# Autodesk Inventor assembly: MK4n Master Structure
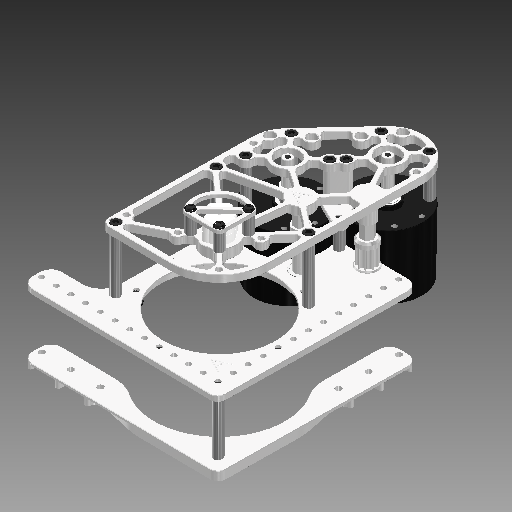
[picture p0: Inventor's stored thumbnail of the model, 512x512]
Saved by Autodesk Inventor 2025 (Build 290162010, 162A)
## iProperties
Created: 2024-07-31
Part Number: MK4n Master Structure
Document SubType Name: Assembly
Designer: rohan
Author: rohan
## Documents named in this file (27)
- D:\ultimate-hecker\Computer-Aided-Design\FRC-Offseason-Design-Training\Parts Library\Drivetrains\Swerve Modules\MK4n\MK4n Master Structure.iam
- D:\ultimate-hecker\Computer-Aided-Design\FRC-Offseason-Design-Training\Parts Library\Drivetrains\Swerve Modules\MK4i\MK4i Wheel Guard.ipt
- D:\ultimate-hecker\Computer-Aided-Design\FRC-Offseason-Design-Training\Parts Library\Drivetrains\Swerve Modules\MK4n\MK4n Midsection.ipt
- D:\ultimate-hecker\Computer-Aided-Design\FRC-Offseason-Design-Training\Parts Library\Drivetrains\Swerve Modules\MK4n\MK4n Motor Mount.ipt
- D:\ultimate-hecker\Computer-Aided-Design\FRC-Offseason-Design-Training\Parts Library\Hardware\Spacers\Spacers & Standoffs\Aluminum Unthreaded Spacer (No. 10 x 1.875Lg x 0.313OD).ipt
- D:\ultimate-hecker\Computer-Aided-Design\FRC-Offseason-Design-Training\Parts Library\Hardware\Spacers\Spacers & Standoffs.ipt
- D:\ultimate-hecker\Computer-Aided-Design\FRC-Offseason-Design-Training\Parts Library\Hardware\Fasteners\Machine Screws\10-32 UNFx2.25 Socket Head Cap Screw.ipt
- D:\ultimate-hecker\Computer-Aided-Design\FRC-Offseason-Design-Training\Parts Library\Hardware\Fasteners\Machine Screws.ipt
- D:\ultimate-hecker\Computer-Aided-Design\FRC-Offseason-Design-Training\Parts Library\Hardware\Spacers\Spacers & Standoffs\Aluminum Unthreaded Spacer (No. 10 x 1.125Lg x 0.313OD).ipt
- D:\ultimate-hecker\Computer-Aided-Design\FRC-Offseason-Design-Training\Parts Library\Hardware\Spacers\Spacers & Standoffs\Aluminum Unthreaded Spacer (No. 10 x 0.625Lg x 0.313OD).ipt
- D:\ultimate-hecker\Computer-Aided-Design\FRC-Offseason-Design-Training\Parts Library\Drivetrains\Swerve Modules\MK4n\MK4n Double Spacer Adapter.ipt
- D:\ultimate-hecker\Computer-Aided-Design\FRC-Offseason-Design-Training\Parts Library\Drivetrains\Swerve Modules\MK4n\MK4n Double Spacer.ipt
- D:\ultimate-hecker\Computer-Aided-Design\FRC-Offseason-Design-Training\Parts Library\Motors\FRC\NEO.ipt
- D:\ultimate-hecker\Computer-Aided-Design\FRC-Offseason-Design-Training\Parts Library\Hardware\Fasteners\Machine Screws\10-32 UNFx1.5 Socket Head Cap Screw.ipt
- D:\ultimate-hecker\Computer-Aided-Design\FRC-Offseason-Design-Training\Parts Library\Hardware\Fasteners\Machine Screws\10-32 UNFx1 Socket Head Cap Screw.ipt
- D:\ultimate-hecker\Computer-Aided-Design\FRC-Offseason-Design-Training\Parts Library\Power Transfer\Bearings and Bushings\Bearings\R188ZZ Bearing.ipt
- D:\ultimate-hecker\Computer-Aided-Design\FRC-Offseason-Design-Training\Parts Library\Drivetrains\Swerve Modules\MK4i\MK4i Steering Shaft Spacer.ipt
- D:\ultimate-hecker\Computer-Aided-Design\FRC-Offseason-Design-Training\Parts Library\Drivetrains\Swerve Modules\MK4i\MK4i Steering Shaft.ipt
- D:\ultimate-hecker\Computer-Aided-Design\FRC-Offseason-Design-Training\Parts Library\Power Transfer\Bearings and Bushings\Bearings\688 Bearing.ipt
- D:\ultimate-hecker\Computer-Aided-Design\FRC-Offseason-Design-Training\Parts Library\Hardware\Spacers\Spacers & Standoffs\SDS Neo Shaft Spacer 0.5mm.ipt
- D:\ultimate-hecker\Computer-Aided-Design\FRC-Offseason-Design-Training\Parts Library\Hardware\Spacers\Spacers & Standoffs\SDS Neo Shaft Spacer 0.437.ipt
- D:\ultimate-hecker\Computer-Aided-Design\FRC-Offseason-Design-Training\Parts Library\Drivetrains\Swerve Modules\MK4i\MK4i Drive Shaft Idler.ipt
- D:\ultimate-hecker\Computer-Aided-Design\FRC-Offseason-Design-Training\Parts Library\Hardware\Spacers\Spacers & Standoffs\Aluminum Unthreaded Spacer (No. 10 x 0.563Lg x 0.313OD).ipt
- D:\ultimate-hecker\Computer-Aided-Design\FRC-Offseason-Design-Training\Parts Library\Drivetrains\Swerve Modules\MK4i\MK4i Encoder Cover.ipt
- D:\ultimate-hecker\Computer-Aided-Design\FRC-Offseason-Design-Training\Parts Library\Electronics\FRC\Sensors\CTRE Mag Encoder.ipt
- D:\ultimate-hecker\Computer-Aided-Design\FRC-Offseason-Design-Training\Parts Library\Hardware\Fasteners\Machine Screws\8-32 UNCx0.875 Button Head Cap Screw.ipt
- D:\ultimate-hecker\Computer-Aided-Design\FRC-Offseason-Design-Training\Parts Library\Hardware\Fasteners\Machine Screws\10-32 UNFx0.25 Button Head Cap Screw.ipt
## Components (49 placed, 24 different names)
1. MK4i Wheel Guard:1 — Insert:1, Insert:11, Flush:1
2. MK4n Midsection:1 — Insert:2, Insert:3, Insert:5, Insert:7, Insert:19, Insert:32, Insert:33, Insert:37, Flush:1, Insert:50, Insert:51, Insert:52, Insert:53, Insert:54
3. MK4n Motor Mount:1 — Insert:4, Insert:6, Insert:8, Insert:9, Insert:10, Insert:12, Insert:13, Insert:14, Insert:15, Insert:20, Insert:21, Insert:26, Insert:27, Insert:28, Insert:29, Insert:30, Insert:31, Insert:34, Insert:38, Insert:40, Insert:41, Insert:42, Insert:45, Insert:46
4. Aluminum Unthreaded Spacer (No. 10 x 1.875Lg x 0.313OD):1 — Insert:3, Insert:4
5. Aluminum Unthreaded Spacer (No. 10 x 1.875Lg x 0.313OD):2 — Insert:5, Insert:6
6. Aluminum Unthreaded Spacer (No. 10 x 1.875Lg x 0.313OD):3 — Insert:1, Insert:2
7. Aluminum Unthreaded Spacer (No. 10 x 1.875Lg x 0.313OD):6 — Insert:7
8. 10-32 UNFx2.25 Socket Head Cap Screw:1 — Insert:8
9. 10-32 UNFx2.25 Socket Head Cap Screw:2 — Insert:9
10. 10-32 UNFx2.25 Socket Head Cap Screw:3 — Insert:11
11. 10-32 UNFx2.25 Socket Head Cap Screw:4 — Insert:10
12. Aluminum Unthreaded Spacer (No. 10 x 1.125Lg x 0.313OD):7 — Insert:12
13. Aluminum Unthreaded Spacer (No. 10 x 1.125Lg x 0.313OD):8 — Insert:14, Insert:25
14. Aluminum Unthreaded Spacer (No. 10 x 1.125Lg x 0.313OD):9 — Insert:13, Insert:22
15. Aluminum Unthreaded Spacer (No. 10 x 1.125Lg x 0.313OD):10 — Insert:15, Insert:24
16. Aluminum Unthreaded Spacer (No. 10 x 0.625Lg x 0.313OD):11 — Insert:18, Insert:19
17. MK4n Double Spacer Adapter:1 — Insert:16, Insert:17, Insert:18, Insert:23
18. MK4n Double Spacer:1 — Insert:16, Insert:17, Insert:20, Insert:21
19. NEO:1 — Insert:22, Insert:23, Insert:35
20. NEO:2 — Insert:24, Insert:25, Insert:36
21. 10-32 UNFx1.5 Socket Head Cap Screw:5 — Insert:30
22. 10-32 UNFx1.5 Socket Head Cap Screw:6 — Insert:31
23. 10-32 UNFx1.5 Socket Head Cap Screw:7 — Insert:28
24. 10-32 UNFx1.5 Socket Head Cap Screw:8 — Insert:29
25. 10-32 UNFx1.5 Socket Head Cap Screw:9 — Insert:26
26. 10-32 UNFx1.5 Socket Head Cap Screw:10 — Insert:27
27. 10-32 UNFx1 Socket Head Cap Screw:11 — Insert:32
28. R188ZZ Bearing:1 — Insert:33, Mate:1
29. MK4i Steering Shaft Spacer:1 — Mate:2
30. MK4i Steering Shaft:1 — Mate:1, Mate:2
31. 688 Bearing:1 — Insert:34
32. SDS Neo Shaft Spacer 0.5mm:12 — Insert:35
33. SDS Neo Shaft Spacer 0.437:13 — Insert:36
34. 688 Bearing:2 — Insert:37, Insert:39
35. 688 Bearing:3 — Insert:38
36. MK4i Drive Shaft Idler:1 — Insert:39
37. Aluminum Unthreaded Spacer (No. 10 x 0.563Lg x 0.313OD):17 — Insert:42
38. Aluminum Unthreaded Spacer (No. 10 x 0.563Lg x 0.313OD):18 — Insert:41, Insert:43
39. Aluminum Unthreaded Spacer (No. 10 x 0.563Lg x 0.313OD):19 — Insert:40, Insert:44
40. MK4i Encoder Cover:1 — Insert:43, Insert:44, Insert:47, Insert:48, Insert:49
41. CTRE Mag Encoder:1 — Insert:45, Insert:46
42. 8-32 UNCx0.875 Button Head Cap Screw:12 — Insert:49
43. 8-32 UNCx0.875 Button Head Cap Screw:13 — Insert:48
44. 8-32 UNCx0.875 Button Head Cap Screw:14 — Insert:47
45. 10-32 UNFx0.25 Button Head Cap Screw:15 — Insert:50
46. 10-32 UNFx0.25 Button Head Cap Screw:16 — Insert:52
47. 10-32 UNFx0.25 Button Head Cap Screw:17 — Insert:54
48. 10-32 UNFx0.25 Button Head Cap Screw:18 — Insert:51
49. 10-32 UNFx0.25 Button Head Cap Screw:19 — Insert:53
## Relationships (57: Insert 54, Mate 2, Flush 1)
- Insert:1: MK4i Wheel Guard:1 ↔ Aluminum Unthreaded Spacer (No. 10 x 1.875Lg x 0.313OD):3
- Insert:2: MK4n Midsection:1 ↔ Aluminum Unthreaded Spacer (No. 10 x 1.875Lg x 0.313OD):3
- Insert:3: MK4n Midsection:1 ↔ Aluminum Unthreaded Spacer (No. 10 x 1.875Lg x 0.313OD):1
- Insert:4: MK4n Motor Mount:1 ↔ Aluminum Unthreaded Spacer (No. 10 x 1.875Lg x 0.313OD):1
- Insert:5: MK4n Midsection:1 ↔ Aluminum Unthreaded Spacer (No. 10 x 1.875Lg x 0.313OD):2
- Insert:6: MK4n Motor Mount:1 ↔ Aluminum Unthreaded Spacer (No. 10 x 1.875Lg x 0.313OD):2
- Insert:7: MK4n Midsection:1 ↔ Aluminum Unthreaded Spacer (No. 10 x 1.875Lg x 0.313OD):6
- Insert:8: MK4n Motor Mount:1 ↔ 10-32 UNFx2.25 Socket Head Cap Screw:1
- Insert:9: MK4n Motor Mount:1 ↔ 10-32 UNFx2.25 Socket Head Cap Screw:2
- Insert:10: MK4n Motor Mount:1 ↔ 10-32 UNFx2.25 Socket Head Cap Screw:4
- Insert:11: MK4i Wheel Guard:1 ↔ 10-32 UNFx2.25 Socket Head Cap Screw:3
- Insert:12: MK4n Motor Mount:1 ↔ Aluminum Unthreaded Spacer (No. 10 x 1.125Lg x 0.313OD):7
- Insert:13: MK4n Motor Mount:1 ↔ Aluminum Unthreaded Spacer (No. 10 x 1.125Lg x 0.313OD):9
- Insert:14: MK4n Motor Mount:1 ↔ Aluminum Unthreaded Spacer (No. 10 x 1.125Lg x 0.313OD):8
- Insert:15: MK4n Motor Mount:1 ↔ Aluminum Unthreaded Spacer (No. 10 x 1.125Lg x 0.313OD):10
- Insert:16: MK4n Double Spacer Adapter:1 ↔ MK4n Double Spacer:1
- Insert:17: MK4n Double Spacer Adapter:1 ↔ MK4n Double Spacer:1
- Insert:18: Aluminum Unthreaded Spacer (No. 10 x 0.625Lg x 0.313OD):11 ↔ MK4n Double Spacer Adapter:1
- Insert:19: MK4n Midsection:1 ↔ Aluminum Unthreaded Spacer (No. 10 x 0.625Lg x 0.313OD):11
- Insert:20: MK4n Motor Mount:1 ↔ MK4n Double Spacer:1
- Insert:21: MK4n Motor Mount:1 ↔ MK4n Double Spacer:1
- Insert:22: Aluminum Unthreaded Spacer (No. 10 x 1.125Lg x 0.313OD):9 ↔ NEO:1
- Insert:23: MK4n Double Spacer Adapter:1 ↔ NEO:1
- Insert:24: Aluminum Unthreaded Spacer (No. 10 x 1.125Lg x 0.313OD):10 ↔ NEO:2
- Insert:25: Aluminum Unthreaded Spacer (No. 10 x 1.125Lg x 0.313OD):8 ↔ NEO:2
- Insert:26: MK4n Motor Mount:1 ↔ 10-32 UNFx1.5 Socket Head Cap Screw:9
- Insert:27: MK4n Motor Mount:1 ↔ 10-32 UNFx1.5 Socket Head Cap Screw:10
- Insert:28: MK4n Motor Mount:1 ↔ 10-32 UNFx1.5 Socket Head Cap Screw:7
- Insert:29: MK4n Motor Mount:1 ↔ 10-32 UNFx1.5 Socket Head Cap Screw:8
- Insert:30: MK4n Motor Mount:1 ↔ 10-32 UNFx1.5 Socket Head Cap Screw:5
- Insert:31: MK4n Motor Mount:1 ↔ 10-32 UNFx1.5 Socket Head Cap Screw:6
- Insert:32: MK4n Midsection:1 ↔ 10-32 UNFx1 Socket Head Cap Screw:11
- Insert:33: MK4n Midsection:1 ↔ R188ZZ Bearing:1
- Insert:34: MK4n Motor Mount:1 ↔ 688 Bearing:1
- Mate:1: R188ZZ Bearing:1 ↔ MK4i Steering Shaft:1
- Mate:2: MK4i Steering Shaft Spacer:1 ↔ MK4i Steering Shaft:1
- Insert:35: NEO:1 ↔ SDS Neo Shaft Spacer 0.5mm:12
- Insert:36: NEO:2 ↔ SDS Neo Shaft Spacer 0.437:13
- Insert:37: MK4n Midsection:1 ↔ 688 Bearing:2
- Insert:38: MK4n Motor Mount:1 ↔ 688 Bearing:3
- Insert:39: 688 Bearing:2 ↔ MK4i Drive Shaft Idler:1
- Insert:40: MK4n Motor Mount:1 ↔ Aluminum Unthreaded Spacer (No. 10 x 0.563Lg x 0.313OD):19
- Insert:41: MK4n Motor Mount:1 ↔ Aluminum Unthreaded Spacer (No. 10 x 0.563Lg x 0.313OD):18
- Insert:42: MK4n Motor Mount:1 ↔ Aluminum Unthreaded Spacer (No. 10 x 0.563Lg x 0.313OD):17
- Insert:43: Aluminum Unthreaded Spacer (No. 10 x 0.563Lg x 0.313OD):18 ↔ MK4i Encoder Cover:1
- Flush:1: MK4i Wheel Guard:1 ↔ MK4n Midsection:1
- Insert:44: Aluminum Unthreaded Spacer (No. 10 x 0.563Lg x 0.313OD):19 ↔ MK4i Encoder Cover:1
- Insert:45: MK4n Motor Mount:1 ↔ CTRE Mag Encoder:1
- Insert:46: MK4n Motor Mount:1 ↔ CTRE Mag Encoder:1
- Insert:47: MK4i Encoder Cover:1 ↔ 8-32 UNCx0.875 Button Head Cap Screw:14
- Insert:48: MK4i Encoder Cover:1 ↔ 8-32 UNCx0.875 Button Head Cap Screw:13
- Insert:49: MK4i Encoder Cover:1 ↔ 8-32 UNCx0.875 Button Head Cap Screw:12
- Insert:50: MK4n Midsection:1 ↔ 10-32 UNFx0.25 Button Head Cap Screw:15
- Insert:51: MK4n Midsection:1 ↔ 10-32 UNFx0.25 Button Head Cap Screw:18
- Insert:52: MK4n Midsection:1 ↔ 10-32 UNFx0.25 Button Head Cap Screw:16
- Insert:53: MK4n Midsection:1 ↔ 10-32 UNFx0.25 Button Head Cap Screw:19
- Insert:54: MK4n Midsection:1 ↔ 10-32 UNFx0.25 Button Head Cap Screw:17
